# Autodesk Inventor assembly: ensemble
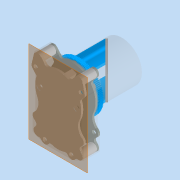
[picture p0: Inventor's stored thumbnail of the model, 180x180]
Saved by Autodesk Inventor 2022 (Build 260153000, 153)
## iProperties
Created: 2022-07-29
Part Number: ensemble
Document SubType Name: Assembly
Designer: andre
Author: andre
## Documents named in this file (7)
- C:\Users\andre\3D Objects\lidar\CAD_inventor\ensemble.iam
- C:\Users\andre\3D Objects\lidar\CAD_inventor\top_plate.ipt
- C:\Users\andre\3D Objects\lidar\CAD_inventor\gear.ipt
- C:\Users\andre\3D Objects\lidar\CAD_inventor\mirror_holder.ipt
- C:\Users\andre\3D Objects\lidar\CAD_inventor\gear_top_ring.ipt
- C:\Users\andre\3D Objects\lidar\CAD_inventor\bottom_plate.ipt
- C:\Users\andre\3D Objects\lidar\CAD_inventor\simple_lidar_shape.ipt
## Components (6 placed, 6 different names)
1. top_plate:1 — Placage:1, Placage:2, Affleurement:2, Affleurement:3
2. gear:1 — Placage:1, Placage:2, Affleurement:1, Placage:3, Placage:4
3. mirror_holder:1 — Affleurement:1, Placage:3, Placage:4
4. gear_top_ring:1 — Affleurement:2
5. bottom_plate:1 — Affleurement:4, Affleurement:5, Affleurement:6, Affleurement:7
6. simple_lidar_shape:1 — Affleurement:6, Affleurement:7
## Relationships (11: Flush 7, Mate 4)
- Placage:1 [Mate]: top_plate:1 ↔ gear:1
- Placage:2 [Mate]: top_plate:1 ↔ gear:1
- Affleurement:1 [Flush]: gear:1 ↔ mirror_holder:1
- Placage:3 [Mate]: gear:1 ↔ mirror_holder:1
- Placage:4 [Mate]: gear:1 ↔ mirror_holder:1
- Affleurement:2 [Flush]: top_plate:1 ↔ gear_top_ring:1
- Affleurement:3 [Flush] (12 mm): top_plate:1
- Affleurement:4 [Flush]: bottom_plate:1
- Affleurement:5 [Flush]: bottom_plate:1
- Affleurement:6 [Flush]: bottom_plate:1 ↔ simple_lidar_shape:1
- Affleurement:7 [Flush]: bottom_plate:1 ↔ simple_lidar_shape:1
